# Autodesk Inventor assembly: Marker Changer - Slidey Parts
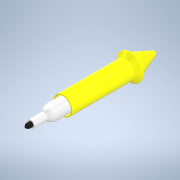
[picture p0: Inventor's stored thumbnail of the model, 180x180]
Saved by Autodesk Inventor 2022.2 (Build 262287000, 287)
## iProperties
Created: 2022-02-09
Part Number: Marker Changer - Slidey Parts
Document SubType Name: Assembly
Designer: smiku
Author: smiku
## Documents named in this file (3)
- C:\Users\smiku\3D Objects\GrabCAD\AACC Mechatonics Capstone\Marker Changer\Subassemblies\Marker Changer - Slidey Parts.iam
- C:\Users\smiku\3D Objects\GrabCAD\AACC Mechatonics Capstone\Marker Changer\Static Marker Barrel.ipt
- C:\Users\smiku\3D Objects\GrabCAD\AACC Mechatonics Capstone\Interface\Marker\Expo Marker Bullet Point.ipt
## Components (2 placed, 2 different names)
1. Static Marker Barrel:4 — Rigid:12
2. Expo Marker Bullet Point:4 — Rigid:12
## Relationships (1: WeldJoint 1)
- Rigid:12 [WeldJoint]: Static Marker Barrel:4 ↔ Expo Marker Bullet Point:4
